# Autodesk Inventor assembly: steelSlides3.0
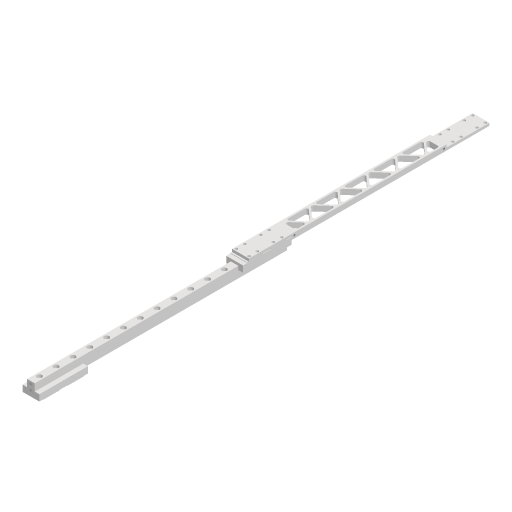
[picture p0: Inventor's stored thumbnail of the model, 512x512]
Saved by Autodesk Inventor 2023 (Build 270158000, 158)
## iProperties
Created: 2022-09-16
Part Number: steelSlides3.0
Document SubType Name: Assembly
Designer: deli
Author: deli
## Documents named in this file (4)
- C:\Users\deli\OneDrive - Eastside Preparatory School\FTC\8103-power-play\CAD\steelSlides3.0.iam
- C:\Users\deli\OneDrive - Eastside Preparatory School\FTC\8103-power-play\CAD\Rail.ipt
- C:\Users\deli\OneDrive - Eastside Preparatory School\FTC\8103-power-play\CAD\Carrige.ipt
- C:\Users\deli\OneDrive - Eastside Preparatory School\FTC\8103-power-play\CAD\Connector Plate.ipt
## Components (7 placed, 3 different names)
1. Rail:1 — Mate:1, Mate:2, Mate:3, Mate:4, Flush:5, Flush:6, Mate:23, Flush:7
2. Carrige:1 — Mate:2, Mate:3, Mate:5, Mate:20, Mate:21, Mate:22, Flush:6
3. Carrige:2 — Mate:1, Mate:4, Mate:5
4. Carrige:3 — Mate:17, Flush:3, Flush:8, Flush:9
5. Carrige:4 — Mate:17, Mate:18, Mate:19, Flush:3, Flush:8
6. Connector Plate:2 — Mate:20, Mate:21, Mate:22
7. Rail:2 — Mate:18, Mate:19, Flush:5, Mate:23, Flush:7, Flush:9
## Relationships (18: Mate 12, Flush 6)
- Mate:1: Rail:1 ↔ Carrige:2
- Mate:2: Rail:1 ↔ Carrige:1
- Mate:3: Rail:1 ↔ Carrige:1
- Mate:4: Rail:1 ↔ Carrige:2
- Mate:5: Carrige:1 ↔ Carrige:2
- Mate:17: Carrige:3 ↔ Carrige:4
- Mate:18: Carrige:4 ↔ Rail:2
- Mate:19: Carrige:4 ↔ Rail:2
- Flush:3: Carrige:3 ↔ Carrige:4
- Mate:20: Carrige:1 ↔ Connector Plate:2
- Mate:21: Carrige:1 ↔ Connector Plate:2
- Mate:22: Carrige:1 ↔ Connector Plate:2
- Flush:5: Rail:1 ↔ Rail:2
- Flush:6 (-242.2 mm): Rail:1 ↔ Carrige:1
- Mate:23: Rail:1 ↔ Rail:2
- Flush:7: Rail:1 ↔ Rail:2
- Flush:8: Carrige:3 ↔ Carrige:4
- Flush:9: Carrige:3 ↔ Rail:2
## Named parameters: stroke = 242.2 mm
